# Autodesk Inventor assembly: Rb PEEK
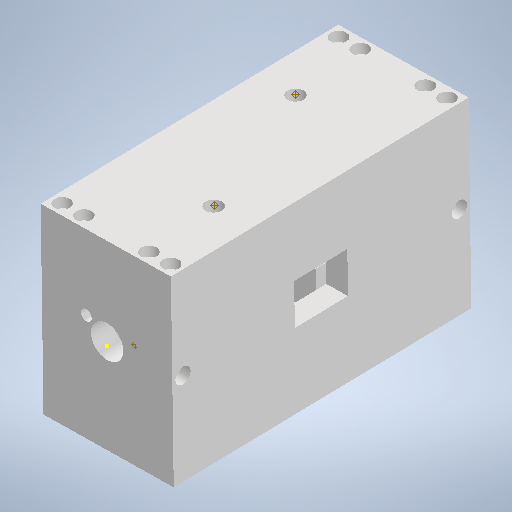
[picture p0: Inventor's stored thumbnail of the model, 512x512]
Saved by Autodesk Inventor 2025.1 (Build 291241000, 241)
## iProperties
Created: 2025-05-09
Part Number: Rb PEEK
Document SubType Name: Assembly
Designer: E. Moreno
Author: E. Moreno
Title: Rb PEEK - Ensamblado
## Documents named in this file (7)
- C:\Users\dell 5810\Documents\M\GitHub\LAFriOC\Rb oven\Rb PEEK\Rb PEEK.iam
- C:\Users\dell 5810\Documents\M\GitHub\LAFriOC\Rb oven\Rb PEEK\Rb PEEK - Arriba.ipt
- C:\Users\dell 5810\Documents\M\GitHub\LAFriOC\Rb oven\Rb PEEK\Rb PEEK - Largo.ipt
- C:\Users\dell 5810\Documents\M\GitHub\LAFriOC\Rb oven\Rb PEEK\Rb PEEK - Corto con ventana.ipt
- C:\Users\dell 5810\Documents\M\GitHub\LAFriOC\Rb oven\Rb PEEK\Rb PEEK - Largo_MIR.ipt
- C:\Users\dell 5810\Documents\M\GitHub\LAFriOC\Rb oven\Rb PEEK\Rb PEEK - Soporte.ipt
- C:\Users\dell 5810\Documents\M\GitHub\LAFriOC\Rb oven\Rb PEEK\Rb PEEK - Abajo.ipt
## Components (8 placed, 6 different names)
1. Rb PEEK - Arriba:1 — Coincidencia:1, Coincidencia:2, Coincidencia:3, Coincidencia:5, Coincidencia:11, Coincidencia:12, Coincidencia:31
2. Rb PEEK - Largo:1 — Coincidencia:1, Coincidencia:2, Coincidencia:3, Coincidencia:4, Coincidencia:18, Coincidencia:20, Coincidencia:21, Coincidencia:22, Coincidencia:23
3. Rb PEEK - Corto con ventana:1 — Coincidencia:4, Coincidencia:5
4. Rb PEEK - Largo_MIR:1 — Coincidencia:11, Coincidencia:12, Coincidencia:26, Coincidencia:27, Coincidencia:28, Coincidencia:32
5. Rb PEEK - Soporte:1 — Coincidencia:29
6. Rb PEEK - Soporte:2 — Coincidencia:30
7. Rb PEEK - Corto con ventana:2 — Coincidencia:18, Coincidencia:20, Coincidencia:31, Coincidencia:32
8. Rb PEEK - Abajo:1 — Coincidencia:21, Coincidencia:22, Coincidencia:23, Coincidencia:26, Coincidencia:27, Coincidencia:28, Coincidencia:29, Coincidencia:30
## Relationships (19: Mate 19)
- Coincidencia:1 [Mate]: Rb PEEK - Arriba:1 ↔ Rb PEEK - Largo:1
- Coincidencia:2 [Mate]: Rb PEEK - Arriba:1 ↔ Rb PEEK - Largo:1
- Coincidencia:3 [Mate]: Rb PEEK - Arriba:1 ↔ Rb PEEK - Largo:1
- Coincidencia:4 [Mate]: Rb PEEK - Largo:1 ↔ Rb PEEK - Corto con ventana:1
- Coincidencia:5 [Mate]: Rb PEEK - Arriba:1 ↔ Rb PEEK - Corto con ventana:1
- Coincidencia:11 [Mate]: Rb PEEK - Arriba:1 ↔ Rb PEEK - Largo_MIR:1
- Coincidencia:12 [Mate]: Rb PEEK - Arriba:1 ↔ Rb PEEK - Largo_MIR:1
- Coincidencia:18 [Mate]: Rb PEEK - Largo:1 ↔ Rb PEEK - Corto con ventana:2
- Coincidencia:20 [Mate]: Rb PEEK - Largo:1 ↔ Rb PEEK - Corto con ventana:2
- Coincidencia:21 [Mate]: Rb PEEK - Largo:1 ↔ Rb PEEK - Abajo:1
- Coincidencia:22 [Mate]: Rb PEEK - Largo:1 ↔ Rb PEEK - Abajo:1
- Coincidencia:23 [Mate]: Rb PEEK - Largo:1 ↔ Rb PEEK - Abajo:1
- Coincidencia:26 [Mate]: Rb PEEK - Largo_MIR:1 ↔ Rb PEEK - Abajo:1
- Coincidencia:27 [Mate]: Rb PEEK - Largo_MIR:1 ↔ Rb PEEK - Abajo:1
- Coincidencia:28 [Mate]: Rb PEEK - Largo_MIR:1 ↔ Rb PEEK - Abajo:1
- Coincidencia:29 [Mate]: Rb PEEK - Soporte:1 ↔ Rb PEEK - Abajo:1
- Coincidencia:30 [Mate]: Rb PEEK - Soporte:2 ↔ Rb PEEK - Abajo:1
- Coincidencia:31 [Mate]: Rb PEEK - Arriba:1 ↔ Rb PEEK - Corto con ventana:2
- Coincidencia:32 [Mate]: Rb PEEK - Largo_MIR:1 ↔ Rb PEEK - Corto con ventana:2
